# Autodesk Inventor assembly: tensegrity_revolute_joint
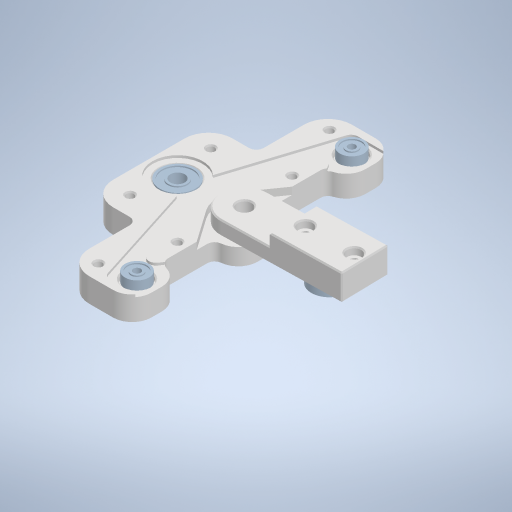
[picture p0: Inventor's stored thumbnail of the model, 512x512]
Saved by Autodesk Inventor 2023.1 (Build 271208000, 208)
## iProperties
Created: 2023-11-21
Part Number: tensegrity_revolute_joint
Document SubType Name: Assembly
Designer: zavrel
Author: zavrel
## Documents named in this file (5)
- C:\Users\zavrel\Documents\_OWNCLOUD_ACTUAL_WORK\_clanek_ustav\Tensegrity_Based_Joionts\03_winding_trajectory\models\tensegrity_revolute_joint.iam
- C:\Users\zavrel\Documents\_OWNCLOUD_ACTUAL_WORK\_clanek_ustav\Tensegrity_Based_Joionts\03_winding_trajectory\models\top.ipt
- C:\Users\zavrel\Documents\_OWNCLOUD_ACTUAL_WORK\_clanek_ustav\Tensegrity_Based_Joionts\03_winding_trajectory\models\bearing_d3D10b4.ipt
- C:\Users\zavrel\Documents\_OWNCLOUD_ACTUAL_WORK\_clanek_ustav\Tensegrity_Based_Joionts\03_winding_trajectory\models\bearing_d6D15b5.ipt
- C:\Users\zavrel\Documents\_OWNCLOUD_ACTUAL_WORK\_clanek_ustav\Tensegrity_Based_Joionts\03_winding_trajectory\models\middle_joint.ipt
## Components (7 placed, 4 different names)
1. top:1 — Rotational:1, Rotational:2, Rotational:3, Rotational:4, Rotational:5
2. bearing_d3D10b4:1 — Rotational:2
3. bearing_d3D10b4:2 — Rotational:1
4. bearing_d6D15b5:1 — Rotational:4
5. bearing_d6D15b5:2
6. bearing_d6D15b5:3 — Rotational:3
7. middle_joint:1 — Rotational:5
## Relationships (5: RevoluteJoint 5)
- Rotational:1 [RevoluteJoint]: top:1 ↔ bearing_d3D10b4:2
- Rotational:2 [RevoluteJoint]: top:1 ↔ bearing_d3D10b4:1
- Rotational:3 [RevoluteJoint]: top:1 ↔ bearing_d6D15b5:3
- Rotational:4 [RevoluteJoint]: top:1 ↔ bearing_d6D15b5:1
- Rotational:5 [RevoluteJoint]: top:1 ↔ middle_joint:1
